# Autodesk Inventor assembly: XYZ Stage V5
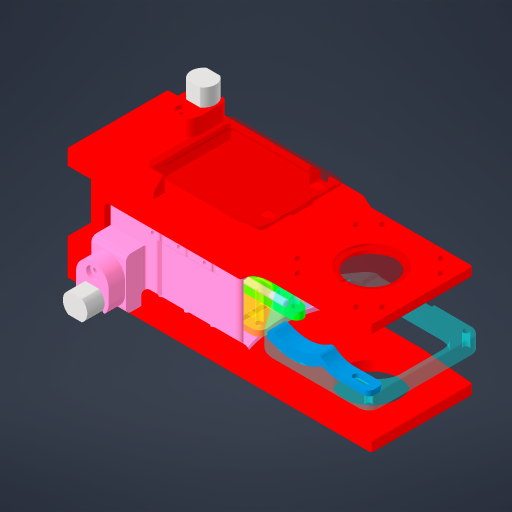
[picture p0: Inventor's stored thumbnail of the model, 512x512]
Saved by Autodesk Inventor 2023.4 (Build 274418000, 418)
## iProperties
Created: 2024-05-20
Part Number: XYZ Stage V5
Document SubType Name: Assembly
Designer: xSibe
Author: xSibe
## Documents named in this file (14)
- C:\.Laptop\.Work\Projects\Project Protocube\Protocube\CAD, STL, OBJ Files\1 CAD\XYZ Stage\XYZ Stage V5.iam
- C:\.Laptop\.Work\Projects\Project Protocube\Protocube\CAD, STL, OBJ Files\1 CAD\XYZ Stage\Z Stage Body V5.ipt
- C:\.Laptop\.Work\Projects\Project Protocube\Protocube\CAD, STL, OBJ Files\1 CAD\XYZ Stage\Z Stage Part V5.ipt
- C:\.Laptop\.Work\Projects\Project Protocube\Protocube\CAD, STL, OBJ Files\1 CAD\XYZ Stage\Y Stage Body v5.ipt
- C:\.Laptop\.Work\Projects\Project Protocube\Protocube\CAD, STL, OBJ Files\1 CAD\XYZ Stage\Y Stage Part V5.ipt
- C:\.Laptop\.Work\Projects\Project Protocube\Protocube\CAD, STL, OBJ Files\1 CAD\XYZ Stage\X Stage Body V5.ipt
- C:\.Laptop\.Work\Projects\Project Protocube\Protocube\CAD, STL, OBJ Files\1 CAD\XYZ Stage\X Stage Part V5.ipt
- C:\.Laptop\.Work\Projects\Project Protocube\Protocube\CAD, STL, OBJ Files\1 CAD\XYZ Stage\X Stage Clamp V5.ipt
- C:\.Laptop\.Work\Projects\Project Protocube\Protocube\CAD, STL, OBJ Files\1 CAD\XYZ Stage\Z Stage Electrical Cover.ipt
- C:\.Laptop\.Work\Projects\Project Protocube\Protocube\CAD, STL, OBJ Files\1 CAD\XYZ Stage\Z Stage Motor Clamp V5.ipt
- C:\.Laptop\.Work\Projects\Project Protocube\Protocube\CAD, STL, OBJ Files\1 CAD\XYZ Stage\DC Motor.ipt
- C:\.Laptop\.Work\Projects\Project Protocube\Protocube\CAD, STL, OBJ Files\1 CAD\XYZ Stage\Y Stage Motor Clamp V5.ipt
- C:\.Laptop\.Work\Projects\Project Protocube\Protocube\CAD, STL, OBJ Files\1 CAD\XYZ Stage\X Stage Motor Clamp V5.ipt
- C:\.Laptop\.Work\Projects\Project Protocube\Protocube\CAD, STL, OBJ Files\1 CAD\XYZ Stage\Z Stage LED Mount V5.ipt
## Components (15 placed, 13 different names)
1. DC Motor:1 — Mate:3, Mate:4, Mate:5
2. DC Motor:2 — Mate:6, Mate:7, Mate:8
3. DC Motor:3 — Mate:9, Mate:10, Mate:11
4. Z Stage Body V5:1 — Mate:3, Mate:4, Mate:5, Mate:12
5. Z Stage Part V5:1 — Mate:2, Mate:6, Mate:7, Mate:8, Mate:13
6. Z Stage LED Mount V5:1
7. Z Stage Electrical Cover:1
8. Z Stage Motor Clamp V5:1 — Mate:12
9. Y Stage Body v5:1 — Mate:2, Mate:9, Mate:10, Mate:11, Mate:14
10. Y Stage Part V5:1
11. Y Stage Motor Clamp V5:1 — Mate:13
12. X Stage Body V5:1 — Mate:15, Mate:16
13. X Stage Part V5:1 — Mate:15, Mate:16
14. X Stage Clamp V5:1
15. X Stage Motor Clamp V5:1 — Mate:14
## Relationships (15: Mate 15)
- Mate:2 (0.375 mm): Z Stage Part V5:1 ↔ Y Stage Body v5:1
- Mate:3: DC Motor:1 ↔ Z Stage Body V5:1
- Mate:4: DC Motor:1 ↔ Z Stage Body V5:1
- Mate:5: DC Motor:1 ↔ Z Stage Body V5:1
- Mate:6: DC Motor:2 ↔ Z Stage Part V5:1
- Mate:7 (0.075 mm): DC Motor:2 ↔ Z Stage Part V5:1
- Mate:8: DC Motor:2 ↔ Z Stage Part V5:1
- Mate:9: DC Motor:3 ↔ Y Stage Body v5:1
- Mate:10 (0.075 mm): DC Motor:3 ↔ Y Stage Body v5:1
- Mate:11: DC Motor:3 ↔ Y Stage Body v5:1
- Mate:12: Z Stage Body V5:1 ↔ Z Stage Motor Clamp V5:1
- Mate:13: Z Stage Part V5:1 ↔ Y Stage Motor Clamp V5:1
- Mate:14: Y Stage Body v5:1 ↔ X Stage Motor Clamp V5:1
- Mate:15: X Stage Body V5:1 ↔ X Stage Part V5:1
- Mate:16: X Stage Body V5:1 ↔ X Stage Part V5:1
